# Autodesk Inventor assembly: handle_monitor
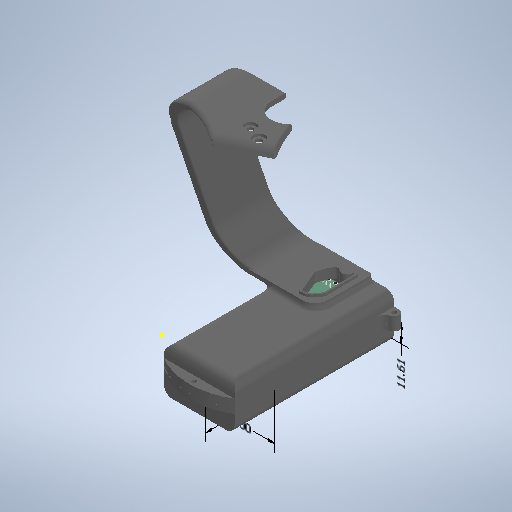
[picture p0: Inventor's stored thumbnail of the model, 512x512]
Saved by Autodesk Inventor 2026.1 (Build 301233020, 233B)
## iProperties
Created: 2026-02-03
Part Number: handle_monitor
Document SubType Name: Assembly
Designer: hibik
Author: hibik
## Documents named in this file (7)
- C:\Users\hibik\Documents\Robomech\HR\controller\hard\handle_right\handle_monitor.iam
- C:\Users\hibik\Documents\Robomech\HR\controller\hard\handle_right\handle_monitor.ipt
- C:\Users\hibik\Documents\Robomech\HR\controller\hard\board\controller_board\controller_board.iam
- C:\Users\hibik\Documents\Robomech\HR\controller\hard\handle_right\battery_box.ipt
- C:\Users\hibik\Documents\Robomech\HR\controller\hard\handle_right\handle_monitor_case_under.ipt
- C:\Users\hibik\Documents\Robomech\HR\controller\hard\handle_right\OLED_Display.iam
- C:\Users\hibik\Documents\Robomech\HR\controller\hard\handle_right\handle_monitor_case_side.ipt
## Components (6 placed, 6 different names)
1. handle_monitor:1 — 挿入:1, 角度:1, フラッシュ:2, メイト:1, フラッシュ:3, 挿入:3, 角度:3
2. controller_board:2 [sub-assembly] — 挿入:1, 角度:1, 挿入:2, 角度:2
3. battery_box:1 — 挿入:2, 角度:2
4. handle_monitor_case_under:1 — フラッシュ:2, メイト:1, フラッシュ:3
5. OLED_Display:1 [sub-assembly] — 挿入:3, 角度:3
6. handle_monitor_case_side:1
## Relationships (9: Insert 3, Angle 3, Flush 2, Mate 1)
- 挿入:1 [Insert]: handle_monitor:1 ↔ controller_board:2
- 角度:1 [Angle] (0 deg): handle_monitor:1 ↔ controller_board:2
- 挿入:2 [Insert]: controller_board:2 ↔ battery_box:1
- 角度:2 [Angle] (0 deg): controller_board:2 ↔ battery_box:1
- フラッシュ:2 [Flush]: handle_monitor:1 ↔ handle_monitor_case_under:1
- メイト:1 [Mate]: handle_monitor:1 ↔ handle_monitor_case_under:1
- フラッシュ:3 [Flush]: handle_monitor:1 ↔ handle_monitor_case_under:1
- 挿入:3 [Insert]: handle_monitor:1 ↔ OLED_Display:1
- 角度:3 [Angle] (0 deg): handle_monitor:1 ↔ OLED_Display:1
